# Autodesk Inventor assembly: Sarax_SAM3
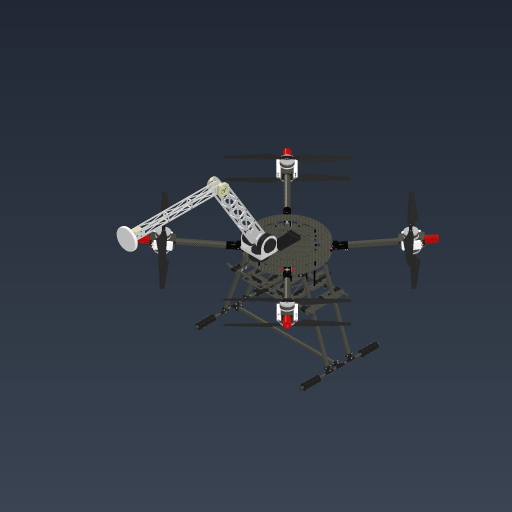
[picture p0: Inventor's stored thumbnail of the model, 512x512]
Saved by Autodesk Inventor 2024.1 (Build 281209000, 209)
## iProperties
Created: 2024-01-12
Part Number: Sarax_SAM3
Document SubType Name: Assembly
Designer: dzw04
Author: dzw04
## Documents named in this file (3)
- C:\Users\dzw04\Saxion\Mechatronica Lectoraat LMECH LED - Database ARG\Component_Database\SARAX\Sarax_SAM3.iam
- C:\Users\dzw04\Saxion\Mechatronica Lectoraat LMECH LED - Database ARG\Component_Database\SARAX\01. CAD\01. 3D_Drawing\Sarax_Quad.iam
- C:\Users\dzw04\Saxion\Mechatronica Lectoraat LMECH LED - Database ARG\Component_Database\SAM3\01. CAD\01. 3D_Drawing\Sam3.iam
## Components (2 placed, 2 different names)
1. Sarax_Quad:1 [sub-assembly] — Mate:1, Mate:2
2. Sam3:1 [sub-assembly] — Mate:1, Mate:2
## Relationships (2: Mate 2)
- Mate:1: Sarax_Quad:1 ↔ Sam3:1
- Mate:2: Sarax_Quad:1 ↔ Sam3:1
